# Autodesk Inventor assembly: chassis weldment center
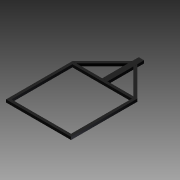
[picture p0: Inventor's stored thumbnail of the model, 180x180]
Saved by Autodesk Inventor 2012 (Build 160160000, 160)
## iProperties
Created: 2011-09-30
Part Number: chassis weldment center
Document SubType Name: Weldment
Designer: Antonella
Weld Material: Welded Aluminum-6061
Author: Antonella
## Documents named in this file (6)
- C:\Users\Antonella\Documents\GCC Robotics 2012 - Mechanical\Robot 2.0\Chassis\chassis weldment center.iam
- C:\Users\Antonella\Documents\GCC Robotics 2012 - Mechanical\Robot 2.0\Chassis\frame member front.ipt
- C:\Users\Antonella\Documents\GCC Robotics 2012 - Mechanical\Robot 2.0\Chassis\frame member side.ipt
- C:\Users\Antonella\Documents\GCC Robotics 2012 - Mechanical\Robot 2.0\Chassis\frame member crossbrace middle.ipt
- C:\Users\Antonella\Documents\GCC Robotics 2012 - Mechanical\Robot 2.0\Chassis\frame member back angle.ipt
- C:\Users\Antonella\Documents\GCC Robotics 2012 - Mechanical\Robot 2.0\Chassis\frame member back center.ipt
## Components (7 placed, 5 different names)
1. frame member front:1 — Mate:1, Flush:1, Mate:2, Mate:3, Flush:2, Mate:4
2. frame member side:1 — Mate:1, Flush:1, Mate:2, Mate:5, Flush:3, Mate:6
3. frame member side:2 — Mate:3, Flush:2, Mate:4
4. frame member crossbrace middle:1 — Mate:5, Flush:3, Mate:6, Mate:7, Flush:4, Mate:9, Flush:5, Mate:11, Flush:6, Mate:12
5. frame member back angle:1 — Mate:7, Flush:4, Mate:14
6. frame member back angle:2 — Mate:9, Flush:5, Mate:13
7. frame member back center:1 — Mate:11, Flush:6, Mate:12, Mate:13, Mate:14
## Relationships (18: Mate 12, Flush 6)
- Mate:1: frame member front:1 ↔ frame member side:1
- Flush:1: frame member front:1 ↔ frame member side:1
- Mate:2: frame member front:1 ↔ frame member side:1
- Mate:3: frame member front:1 ↔ frame member side:2
- Flush:2: frame member front:1 ↔ frame member side:2
- Mate:4: frame member front:1 ↔ frame member side:2
- Mate:5: frame member side:1 ↔ frame member crossbrace middle:1
- Flush:3: frame member side:1 ↔ frame member crossbrace middle:1
- Mate:6: frame member side:1 ↔ frame member crossbrace middle:1
- Mate:7: frame member crossbrace middle:1 ↔ frame member back angle:1
- Flush:4: frame member crossbrace middle:1 ↔ frame member back angle:1
- Mate:9: frame member crossbrace middle:1 ↔ frame member back angle:2
- Flush:5: frame member crossbrace middle:1 ↔ frame member back angle:2
- Mate:11: frame member crossbrace middle:1 ↔ frame member back center:1
- Flush:6: frame member crossbrace middle:1 ↔ frame member back center:1
- Mate:12: frame member crossbrace middle:1 ↔ frame member back center:1
- Mate:13: frame member back angle:2 ↔ frame member back center:1
- Mate:14: frame member back angle:1 ↔ frame member back center:1
